# Autodesk Inventor assembly: AGF
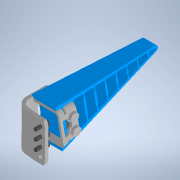
[picture p0: Inventor's stored thumbnail of the model, 180x180]
Saved by Autodesk Inventor 2020 (Build 240168000, 168)
## iProperties
Created: 2020-05-25
Part Number: AGF
Document SubType Name: Assembly
Designer: Gebruiker
Author: Gebruiker
## Documents named in this file (4)
- C:\Users\Gebruiker\Documents\GitHub\BeerMinder\3D-model\servo\AGF.iam
- C:\Users\Gebruiker\Documents\GitHub\BeerMinder\3D-model\servo\AIS2020\3899099 DHAS-MA-B6-80.iam
- C:\Users\Gebruiker\Documents\GitHub\BeerMinder\3D-model\servo\AIS2020\4463570 DHAS-ME-H9-80.iam
- C:\Users\Gebruiker\Documents\GitHub\BeerMinder\3D-model\servo\3998964 DHAS-GF-80-U-BU.ipt
## Components (3 placed, 3 different names)
1. 3899099 DHAS-MA-B6-80:1 [sub-assembly] — Mate:1, Mate:2, Mate:4
2. 4463570 DHAS-ME-H9-80:1 [sub-assembly] — Mate:1, Mate:2, Mate:3, Mate:4, Mate:5, Mate:6
3. 3998964 DHAS-GF-80-U-BU:1 — Mate:3, Mate:5, Mate:6
## Relationships (6: Mate 6)
- Mate:1: 3899099 DHAS-MA-B6-80:1 ↔ 4463570 DHAS-ME-H9-80:1
- Mate:2: 3899099 DHAS-MA-B6-80:1 ↔ 4463570 DHAS-ME-H9-80:1
- Mate:3: 4463570 DHAS-ME-H9-80:1 ↔ 3998964 DHAS-GF-80-U-BU:1
- Mate:4: 3899099 DHAS-MA-B6-80:1 ↔ 4463570 DHAS-ME-H9-80:1
- Mate:5 (-8 mm): 4463570 DHAS-ME-H9-80:1 ↔ 3998964 DHAS-GF-80-U-BU:1
- Mate:6 (-1 mm): 4463570 DHAS-ME-H9-80:1 ↔ 3998964 DHAS-GF-80-U-BU:1
